# Autodesk Inventor assembly: Assembly suelo
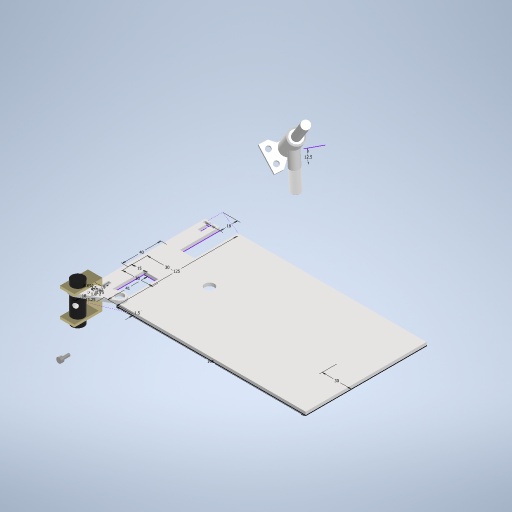
[picture p0: Inventor's stored thumbnail of the model, 512x512]
Saved by Autodesk Inventor 2024 (Build 280153000, 153)
## iProperties
Created: 2023-05-06
Part Number: Assembly suelo
Document SubType Name: Assembly
Designer: Diego
Author: Diego
## Documents named in this file (10)
- C:\Users\Diego\Desktop\Proyecto2_micros\Assembly suelo.iam
- C:\Users\Diego\Desktop\Proyecto2_micros\suelo_imp.ipt
- C:\Users\Diego\Desktop\Proyecto2_micros\tornillo_5_5_10_5.ipt
- C:\Users\Diego\Desktop\Proyecto2_micros\llanta_1.ipt
- C:\Users\Diego\Desktop\Proyecto2_micros\tornillo_7_21.ipt
- C:\Users\Diego\Desktop\Proyecto2_micros\movil_llanta.ipt
- C:\Users\Diego\Desktop\Proyecto2_micros\conex_llantamov.ipt
- C:\Users\Diego\Desktop\Proyecto2_micros\soporte1.ipt
- C:\Users\Diego\Desktop\Proyecto2_micros\barra_volante.ipt
- C:\Users\Diego\Desktop\Proyecto2_micros\union_movllantas.ipt
## Components (9 placed, 9 different names)
1. suelo_imp:1 — Rigid:3, Rotational:1, Rotation:1
2. tornillo_5_5_10_5:1
3. llanta_1:1 — Rotational:1, Cylindrical:1
4. tornillo_7_21:1 — Rigid:3
5. movil_llanta:1 — Cylindrical:1, Rigid:4
6. conex_llantamov:1 — Rigid:4
7. soporte1:1 — Cylindrical:2, Rotation:1
8. barra_volante:1 — Cylindrical:2, Rigid:5
9. union_movllantas:1 — Rigid:5
## Relationships (7: WeldJoint 3, CylindricalJoint 2, RevoluteJoint 1, RelateRotation 1)
- Rigid:3 [WeldJoint]: suelo_imp:1 ↔ tornillo_7_21:1
- Rotational:1 [RevoluteJoint]: suelo_imp:1 ↔ llanta_1:1
- Cylindrical:1: llanta_1:1 ↔ movil_llanta:1
- Rigid:4 [WeldJoint] (12 mm): movil_llanta:1 ↔ conex_llantamov:1
- Cylindrical:2: soporte1:1 ↔ barra_volante:1
- Rotation:1 [RelateRotation] (1 ul): suelo_imp:1 ↔ soporte1:1
- Rigid:5 [WeldJoint]: barra_volante:1 ↔ union_movllantas:1
